# Autodesk Inventor assembly: CAJA_ENGRANAJES_COMPLETA
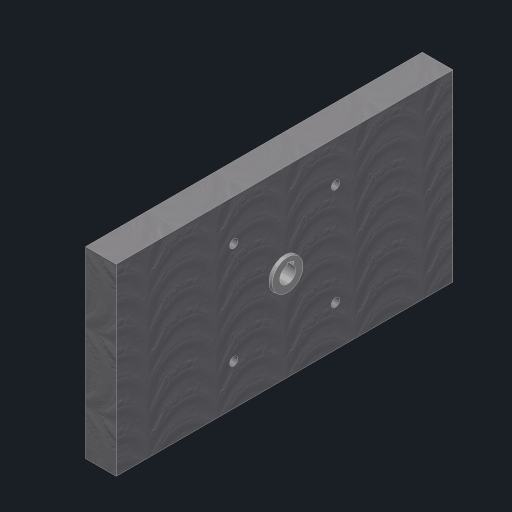
[picture p0: Inventor's stored thumbnail of the model, 512x512]
Saved by Autodesk Inventor 2024.3 (Build 283343000, 343)
## iProperties
Created: 2024-06-29
Part Number: CAJA_ENGRANAJES_COMPLETA
Material: Generic
Document SubType Name: Assembly
Designer: Niler
Author: Niler
## Documents named in this file (4)
- C:\Users\Niler\OneDrive\Escritorio\RECICLADOR\RECICLADOR_MODELO_3D\CAJA_ENGRANAJES\CAJA_ENGRANAJES_COMPLETA.iam
- C:\Users\Niler\OneDrive\Escritorio\RECICLADOR\RECICLADOR_MODELO_3D\CAJA_ENGRANAJES\CAJA.ipt
- C:\Users\Niler\OneDrive\Escritorio\RECICLADOR\RECICLADOR_MODELO_3D\CAJA_ENGRANAJES\ENGRANAJES\Design Accelerator\Spur Gear11.ipt
- C:\Users\Niler\OneDrive\Escritorio\RECICLADOR\RECICLADOR_MODELO_3D\CAJA_ENGRANAJES\ENGRANAJES\Design Accelerator\Spur Gear21.ipt
## Components (4 placed, 3 different names)
1. CAJA:1 — Mate:5, Mate:6, Mate:7, Mate:8
2. Spur Gear2:1 — Flush:2, Mate:6
3. Spur Gear1:1 — Flush:1, Flush:2, Mate:7
4. Spur Gear2:2 — Flush:1, Mate:5, Mate:8
## Relationships (6: Mate 4, Flush 2)
- Flush:1: Spur Gear1:1 ↔ Spur Gear2:2
- Flush:2: Spur Gear2:1 ↔ Spur Gear1:1
- Mate:5: CAJA:1 ↔ Spur Gear2:2
- Mate:6: CAJA:1 ↔ Spur Gear2:1
- Mate:7: CAJA:1 ↔ Spur Gear1:1
- Mate:8: CAJA:1 ↔ Spur Gear2:2
